# Autodesk Inventor assembly: Chassis assembly
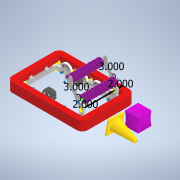
[picture p0: Inventor's stored thumbnail of the model, 180x180]
Saved by Autodesk Inventor 2022 (Build 260153000, 153)
## iProperties
Created: 2022-11-14
Part Number: Chassis assembly
Document SubType Name: Assembly
Designer: s135320
Author: s135320
## Documents named in this file (35)
- D:\Chassis assembly.iam
- D:\Chassis\Chassis side 1.ipt
- D:\Chassis\Chassis side 2.ipt
- D:\STEP Files\Hardware\Gussets\TTB T Gusset\TTB-00012_T-Gusset.ipt
- D:\STEP Files\Bearings\1-2inch Hex Bering\217-3875-STEP-20140818.ipt
- D:\STEP Files\Gearboxes\WCP SS Flipped Gearbox\WCP-0235.iam
- D:\bumper simple.ipt
- D:\bumper bracket.ipt
- D:\1872A111_Slide-Snap Draw Latch.ipt
- D:\bumper bracket - Copy.ipt
- D:\drive hex shaft.ipt
- D:\bumper piece 1.ipt
- D:\Drive spacer.ipt
- D:\WCP-0087.ipt
- D:\STEP Files\Hardware\Shaft Collars\TTB Balanced Hex Collar\TTB-0013_Balanced Half Inch Hex Shaft Collar.ipt
- D:\bumper beam.ipt
- D:\STEP Files\Hardware\teleiscope arm\WCP - Greyt Telescope (Stages 1-4).iam
- D:\Imported Components\am-0940b 6 in HiGrip Wheel\am-0940b 6 in HiGrip Wheel.iam
- D:\Imported Components\am-2568 500EX Hex Hub\am-2568 500EX Hex Hub.ipt
- D:\Robot bottom.ipt
- D:\STEP Files\Electrical\Breaker\am-0282 120a Circuit Breaker.ipt
- D:\STEP Files\Electrical\Power Distribution Hub\REV-11-1850.ipt
- D:\STEP Files\Electrical\Pneumatic Hub\REV-11-1852.ipt
- D:\STEP Files\Electrical\Roborio V2\am-3000a National Instruments roboRIO 2.ipt
- D:\STEP Files\Pnumatics\Compressor\am-3227 Pneumatic Compressor 1.1_Pump REV2.ipt
- D:\STEP Files\Electrical\Battery\ELEC_Battery_NP18-12B.iam
- D:\Intake hex.ipt
- D:\intake-1.ipt
- D:\TTB-0058 5M 15t HTD ALUMINUM PULLEY.ipt
- D:\am-3480 4IN 500Hex Bore Compliant Wheel REV2.ipt
- D:\am-4541 Sushi Roller 500 Hex Bore.ipt
- D:\Intake mount.ipt
- D:\Intake base hex.ipt
- D:\Imported Components\am-4700_bpc Cube\am-4700_bpc Cube.ipt
- D:\Imported Components\am-4700_syc Cone\am-4700_syc Cone.ipt
## Components (171 placed, 34 different names)
1. WCP - Greyt Telescope (Stages 1-4):1 [sub-assembly]
2. bumper simple:1 — Mate:69, Mate:70, Flush:10, Mate:83, Mate:86, Mate:98, Mate:104, Mate:303, Mate:354, Mate:355, Mate:356, Mate:357, Mate:358, Mate:412
3. Intake base hex:1 — Mate:532, Mate:533, Mate:534, Mate:535, Mate:536
4. 217-3875-STEP-20140818:30 — Mate:528, Mate:529, Mate:534
5. 217-3875-STEP-20140818:31 — Mate:530, Mate:531, Mate:532, Mate:533
6. am-4700_bpc Cube:1
7. am-4700_syc Cone:1
8. 217-3875-STEP-20140818:29 — Mate:525, Mate:526
9. 217-3875-STEP-20140818:28 — Mate:524, Mate:527, Mate:535, Mate:536
10. 217-3875-STEP-20140818:27 — Mate:521, Mate:522
11. 217-3875-STEP-20140818:26 — Mate:520, Mate:523
12. Intake mount:2 — Mate:517, Mate:518, Mate:519, Mate:524, Mate:525, Mate:526, Mate:527
13. Intake mount:1 — Mate:514, Mate:515, Mate:516, Mate:520, Mate:521, Mate:522, Mate:523, Mate:537
14. Chassis side 1:1 — Mate:8, Mate:9, Flush:3, Mate:10, Mate:11, Flush:4, Mate:22, Mate:29, Mate:30, Mate:31, Mate:32, Mate:37, Mate:38, Mate:39, Mate:40, Mate:41, Mate:42, Mate:45, Mate:55, Mate:61, Mate:64, Mate:65, Mate:68, Mate:126, Mate:200, Mate:287, Mate:288, Mate:331, Mate:332, Mate:333, Mate:348, Mate:349, Mate:350, Mate:351, Mate:352, Mate:353
15. Chassis side 1:2 — Mate:1, Mate:2, Mate:3, Mate:14, Mate:15, Flush:6, Mate:20, Mate:25, Mate:26, Mate:27, Mate:28, Mate:33, Mate:34, Mate:35, Mate:36, Mate:43, Mate:44, Mate:46, Mate:56, Mate:62, Mate:63, Mate:279, Mate:280, Mate:292, Mate:293, Mate:294, Mate:295, Mate:325, Mate:326, Mate:327, Mate:328, Mate:329, Mate:330, Mate:410, Mate:411
16. Chassis side 2:1 — Mate:12, Mate:13, Flush:5, Mate:21, Flush:9, Mate:23, Mate:24, Mate:57, Mate:58, Mate:59, Mate:60, Mate:69, Mate:70, Mate:87, Mate:88, Mate:99, Mate:100, Mate:291
17. Chassis side 2:2 — Mate:4, Mate:5, Flush:1, Mate:6, Mate:7, Flush:2, Mate:18, Mate:19, Flush:8, Flush:10, Mate:84, Mate:85, Mate:105, Mate:106, Mate:290, Mate:407, Mate:408, Mate:409
18. TTB-00012_T-Gusset:1 — Mate:14, Mate:15, Flush:6, Mate:57
19. TTB-00012_T-Gusset:2 — Mate:1, Mate:2, Mate:3, Mate:4, Mate:5, Flush:1, Mate:56, Mate:407, Mate:517, Mate:518, Mate:519
20. TTB-00012_T-Gusset:3 — Mate:22, Mate:23, Mate:24, Mate:60, Mate:61
21. TTB-00012_T-Gusset:5 — Mate:20, Mate:21, Flush:9, Mate:58, Mate:59
22. TTB-00012_T-Gusset:6 — Mate:6, Mate:7, Flush:2, Mate:8, Mate:9, Flush:3, Mate:55, Mate:290, Mate:514, Mate:515, Mate:516
23. TTB-00012_T-Gusset:7 — Mate:10, Mate:11, Flush:4, Mate:12, Mate:13, Flush:5, Mate:291
24. TTB-00012_T-Gusset:8 — Mate:18, Mate:19, Flush:8
25. 217-3875-STEP-20140818:3 — Mate:37, Mate:38, Mate:197, Mate:198, Mate:406
26. 217-3875-STEP-20140818:4 — Mate:29, Mate:30, Mate:200, Mate:201
27. 217-3875-STEP-20140818:5 — Mate:39, Mate:40, Mate:203, Mate:204, Mate:388
28. 217-3875-STEP-20140818:6 — Mate:35, Mate:36, Mate:208
29. 217-3875-STEP-20140818:8 — Mate:33, Mate:34, Mate:252, Mate:253, Mate:254
30. 217-3875-STEP-20140818:9 — Mate:31, Mate:32, Mate:202
31. 217-3875-STEP-20140818:11 — Mate:27, Mate:28, Mate:385
32. 217-3875-STEP-20140818:12 — Mate:25, Mate:26, Mate:206, Mate:207, Mate:379
33. WCP-0235:1 [sub-assembly] — Mate:43, Mate:44, Mate:46, Mate:362, Mate:364
34. WCP-0235:2 [sub-assembly] — Mate:41, Mate:42, Mate:45, Mate:401, Mate:402
35. 217-3875-STEP-20140818:13 — Mate:62, Mate:63, Mate:382
36. 217-3875-STEP-20140818:14 — Mate:64, Mate:65, Mate:107, Mate:108, Mate:111
37. 217-3875-STEP-20140818:16 — Mate:68, Mate:126, Mate:400
38. bumper bracket:6 — Mate:86, Mate:87
39. 1872A111_Slide-Snap Draw Latch:6 — Mate:88
40. bumper bracket:7 — Mate:83, Mate:85
41. 1872A111_Slide-Snap Draw Latch:7 — Mate:84
42. 1872A111_Slide-Snap Draw Latch:8 — Mate:99
43. bumper bracket - Copy:3 — Mate:98, Mate:100
44. 1872A111_Slide-Snap Draw Latch:9 — Mate:105, Mate:465
45. bumper bracket - Copy:4 — Mate:104, Mate:106, Mate:465
46. drive hex shaft:1 — Mate:107, Mate:108, Mate:109, Mate:110, Mate:112, Mate:113, Mate:115, Mate:116, Flush:11, Mate:398, Mate:399
47. bumper piece 1:1 — Mate:292, Mate:293, Mate:294, Mate:295, Mate:296, Mate:297
48. Drive spacer:1 — Mate:109, Mate:110, Mate:111, Mate:114
49. WCP-0087:1 — Mate:112, Mate:113, Mate:114, Mate:139
50. TTB-0013_Balanced Half Inch Hex Shaft Collar:1 — Mate:115, Mate:116, Flush:11, Mate:139
51. drive hex shaft:2 — Mate:197, Mate:198, Mate:404, Mate:405
52. Drive spacer:3 — Mate:201
53. WCP-0087:2
54. TTB-0013_Balanced Half Inch Hex Shaft Collar:3
55. drive hex shaft:3 — Mate:203, Mate:204, Mate:386, Mate:387
56. Drive spacer:5 — Mate:202
57. WCP-0087:3
58. TTB-0013_Balanced Half Inch Hex Shaft Collar:5
59. drive hex shaft:4 — Mate:206, Mate:207, Mate:377, Mate:378, Flush:19
60. Drive spacer:7 — Mate:208
61. WCP-0087:4
62. TTB-0013_Balanced Half Inch Hex Shaft Collar:7 — Flush:19
63. drive hex shaft:5 — Mate:380, Mate:381, Flush:18
64. Drive spacer:9
65. WCP-0087:5
66. TTB-0013_Balanced Half Inch Hex Shaft Collar:9 — Flush:18
67. drive hex shaft:6 — Mate:252, Mate:253, Mate:383, Mate:384, Flush:17
68. Drive spacer:11 — Mate:254
69. WCP-0087:6
70. TTB-0013_Balanced Half Inch Hex Shaft Collar:11 — Flush:17
71. 217-3875-STEP-20140818:17 — Mate:279, Mate:280, Mate:363
72. 217-3875-STEP-20140818:18 — Mate:287, Mate:288, Mate:403
73. bumper beam:1 — Mate:296, Mate:297, Mate:301, Mate:302
74. 1872A111_Slide-Snap Draw Latch:10 — Mate:301
75. bumper bracket - Copy:5 — Mate:302, Mate:303
76. bumper piece 1:2 — Mate:325, Mate:326
77. bumper beam:2 — Mate:327
78. 1872A111_Slide-Snap Draw Latch:11
79. bumper bracket - Copy:6 — Mate:357
80. bumper piece 1:3 — Mate:328, Mate:329
81. bumper beam:3 — Mate:330
82. 1872A111_Slide-Snap Draw Latch:12
83. bumper bracket - Copy:7 — Mate:358
84. bumper piece 1:4 — Mate:331, Mate:332
85. bumper beam:4 — Mate:333
86. 1872A111_Slide-Snap Draw Latch:13
87. bumper bracket - Copy:8 — Mate:354
88. bumper piece 1:5 — Mate:348, Mate:349
89. bumper beam:5 — Mate:350
90. 1872A111_Slide-Snap Draw Latch:14
91. bumper bracket - Copy:9 — Mate:355
92. bumper piece 1:6 — Mate:351, Mate:352
93. bumper beam:6 — Mate:353
94. 1872A111_Slide-Snap Draw Latch:15
95. bumper bracket - Copy:10 — Mate:356
96. am-0940b 6 in HiGrip Wheel:10 [sub-assembly] — Mate:359, Mate:360, Mate:361
97. am-2568 500EX Hex Hub:9 — Mate:359, Mate:360, Mate:361, Mate:362, Mate:363, Mate:364
98. am-0940b 6 in HiGrip Wheel:11 [sub-assembly]
99. am-2568 500EX Hex Hub:10 — Mate:380, Mate:381, Mate:382
100. am-0940b 6 in HiGrip Wheel:12 [sub-assembly]
101. am-2568 500EX Hex Hub:11 — Mate:377, Mate:378, Mate:379
102. am-0940b 6 in HiGrip Wheel:13 [sub-assembly]
103. am-2568 500EX Hex Hub:12 — Mate:383, Mate:384, Mate:385
104. am-0940b 6 in HiGrip Wheel:14 [sub-assembly]
105. am-2568 500EX Hex Hub:13 — Mate:386, Mate:387, Mate:388
106. am-0940b 6 in HiGrip Wheel:15 [sub-assembly]
107. am-2568 500EX Hex Hub:14 — Mate:401, Mate:402, Mate:403
108. am-0940b 6 in HiGrip Wheel:16 [sub-assembly]
109. am-2568 500EX Hex Hub:15 — Mate:398, Mate:399, Mate:400
110. am-0940b 6 in HiGrip Wheel:17 [sub-assembly]
111. am-2568 500EX Hex Hub:16 — Mate:404, Mate:405, Mate:406
112. TTB-00012_T-Gusset:9 — Mate:408, Mate:409, Mate:410
113. ELEC_Battery_NP18-12B:1 [sub-assembly]
114. am-3227 Pneumatic Compressor 1.1_Pump REV2:1 — Mate:418
115. am-3000a National Instruments roboRIO 2:1 — Mate:413
116. Robot bottom:1 — Mate:411, Mate:412, Mate:413, Mate:415, Mate:416, Mate:417, Mate:418
117. am-0282 120a Circuit Breaker:1 — Mate:417
118. REV-11-1852:1 — Mate:416
119. REV-11-1850:1 — Mate:415
120. TTB-0013_Balanced Half Inch Hex Shaft Collar:15 — Mate:490, Mate:491, Mate:500
121. am-4541 Sushi Roller 500 Hex Bore:32 — Mate:492, Mate:493, Mate:494, Mate:495, Mate:501
122. TTB-0013_Balanced Half Inch Hex Shaft Collar:16 — Mate:497, Mate:498, Mate:499, Flush:22
123. 217-3875-STEP-20140818:25 — Mate:480, Mate:481, Mate:484, Mate:485, Mate:486, Mate:487, Mate:496, Mate:500
124. 217-3875-STEP-20140818:24 — Mate:479, Mate:482, Mate:483, Mate:495, Mate:499, Mate:511, Mate:512
125. am-4541 Sushi Roller 500 Hex Bore:2 — Mate:508, Mate:509, Mate:510
126. intake-1:3 — Mate:479, Mate:480, Mate:481, Mate:482, Mate:486, Mate:487, Mate:501, Mate:510, Mate:512, Mate:530, Mate:531, Mate:537
127. TTB-0013_Balanced Half Inch Hex Shaft Collar:13 — Mate:442, Mate:443, Flush:21, Mate:444
128. TTB-0013_Balanced Half Inch Hex Shaft Collar:12 — Mate:440, Mate:441, Flush:20, Mate:445, Mate:472
129. TTB-0058 5M 15t HTD ALUMINUM PULLEY:2 — Mate:436, Mate:437, Mate:438, Mate:444
130. TTB-0058 5M 15t HTD ALUMINUM PULLEY:1 — Mate:434, Mate:435, Mate:439, Mate:445
131. 217-3875-STEP-20140818:23 — Mate:433, Mate:439, Mate:469, Mate:472, Mate:513
132. 217-3875-STEP-20140818:22 — Mate:431, Mate:432, Mate:438, Mate:475
133. intake-1:2 — Mate:507, Mate:528, Mate:529
134. Intake hex:2 — Mate:433, Mate:434, Mate:435, Mate:440, Mate:441, Flush:20, Mate:469, Mate:484, Mate:485, Mate:490, Mate:491, Mate:496, Mate:502, Mate:503, Mate:504, Mate:505, Mate:508, Mate:509, Mate:513
135. Intake hex:1 — Mate:431, Mate:432, Mate:436, Mate:437, Mate:442, Mate:443, Flush:21, Mate:473, Mate:474, Mate:476, Mate:477, Mate:483, Mate:492, Mate:493, Mate:497, Mate:498, Mate:511, Flush:22
136. am-4541 Sushi Roller 500 Hex Bore:33 — Mate:502, Mate:503, Mate:506, Mate:507
137. am-3480 4IN 500Hex Bore Compliant Wheel REV2:33 — Mate:504, Mate:505, Mate:506
138. am-4541 Sushi Roller 500 Hex Bore:34
139. am-3480 4IN 500Hex Bore Compliant Wheel REV2:34
140. am-4541 Sushi Roller 500 Hex Bore:35
141. am-3480 4IN 500Hex Bore Compliant Wheel REV2:35
142. am-4541 Sushi Roller 500 Hex Bore:36
143. am-3480 4IN 500Hex Bore Compliant Wheel REV2:36
144. am-4541 Sushi Roller 500 Hex Bore:37
145. am-3480 4IN 500Hex Bore Compliant Wheel REV2:37
146. am-4541 Sushi Roller 500 Hex Bore:38
147. am-3480 4IN 500Hex Bore Compliant Wheel REV2:38
148. am-4541 Sushi Roller 500 Hex Bore:39
149. am-3480 4IN 500Hex Bore Compliant Wheel REV2:39
150. am-4541 Sushi Roller 500 Hex Bore:40
151. am-3480 4IN 500Hex Bore Compliant Wheel REV2:40
152. am-4541 Sushi Roller 500 Hex Bore:41
153. am-3480 4IN 500Hex Bore Compliant Wheel REV2:41
154. am-3480 4IN 500Hex Bore Compliant Wheel REV2:8 — Mate:476, Mate:477, Mate:478
155. am-4541 Sushi Roller 500 Hex Bore:23 — Mate:473, Mate:474, Mate:475, Mate:478
156. am-3480 4IN 500Hex Bore Compliant Wheel REV2:25
157. am-4541 Sushi Roller 500 Hex Bore:24
158. am-3480 4IN 500Hex Bore Compliant Wheel REV2:26
159. am-4541 Sushi Roller 500 Hex Bore:25
160. am-3480 4IN 500Hex Bore Compliant Wheel REV2:27
161. am-4541 Sushi Roller 500 Hex Bore:26
162. am-3480 4IN 500Hex Bore Compliant Wheel REV2:28
163. am-4541 Sushi Roller 500 Hex Bore:27
164. am-3480 4IN 500Hex Bore Compliant Wheel REV2:29
165. am-4541 Sushi Roller 500 Hex Bore:28
166. am-3480 4IN 500Hex Bore Compliant Wheel REV2:30
167. am-4541 Sushi Roller 500 Hex Bore:29
168. am-3480 4IN 500Hex Bore Compliant Wheel REV2:31
169. am-4541 Sushi Roller 500 Hex Bore:30
170. am-3480 4IN 500Hex Bore Compliant Wheel REV2:32 — Mate:494
171. am-4541 Sushi Roller 500 Hex Bore:31
## Component patterns: (9 elements, first: am-4541 Sushi Roller 500 Hex Bore:33 + am-3480 4IN 500Hex Bore Compliant Wheel REV2:33), (9 elements, first: am-3480 4IN 500Hex Bore Compliant Wheel REV2:8 + am-4541 Sushi Roller 500 Hex Bore:23)
## Relationships (385: Mate 364, Flush 21)
- Mate:1: Chassis side 1:2 ↔ TTB-00012_T-Gusset:2
- Mate:2: Chassis side 1:2 ↔ TTB-00012_T-Gusset:2
- Mate:3: Chassis side 1:2 ↔ TTB-00012_T-Gusset:2
- Mate:4: Chassis side 2:2 ↔ TTB-00012_T-Gusset:2
- Mate:5: Chassis side 2:2 ↔ TTB-00012_T-Gusset:2
- Flush:1: Chassis side 2:2 ↔ TTB-00012_T-Gusset:2
- Mate:6: Chassis side 2:2 ↔ TTB-00012_T-Gusset:6
- Mate:7: Chassis side 2:2 ↔ TTB-00012_T-Gusset:6
- Flush:2: Chassis side 2:2 ↔ TTB-00012_T-Gusset:6
- Mate:8: Chassis side 1:1 ↔ TTB-00012_T-Gusset:6
- Mate:9: Chassis side 1:1 ↔ TTB-00012_T-Gusset:6
- Flush:3: Chassis side 1:1 ↔ TTB-00012_T-Gusset:6
- Mate:10: Chassis side 1:1 ↔ TTB-00012_T-Gusset:7
- Mate:11: Chassis side 1:1 ↔ TTB-00012_T-Gusset:7
- Flush:4: Chassis side 1:1 ↔ TTB-00012_T-Gusset:7
- Mate:12: Chassis side 2:1 ↔ TTB-00012_T-Gusset:7
- Mate:13: Chassis side 2:1 ↔ TTB-00012_T-Gusset:7
- Flush:5: Chassis side 2:1 ↔ TTB-00012_T-Gusset:7
- Mate:14: Chassis side 1:2 ↔ TTB-00012_T-Gusset:1
- Mate:15: Chassis side 1:2 ↔ TTB-00012_T-Gusset:1
- Flush:6: Chassis side 1:2 ↔ TTB-00012_T-Gusset:1
- Mate:18: Chassis side 2:2 ↔ TTB-00012_T-Gusset:8
- Mate:19: Chassis side 2:2 ↔ TTB-00012_T-Gusset:8
- Flush:8: Chassis side 2:2 ↔ TTB-00012_T-Gusset:8
- Mate:20: Chassis side 1:2 ↔ TTB-00012_T-Gusset:5
- Mate:21: Chassis side 2:1 ↔ TTB-00012_T-Gusset:5
- Flush:9: Chassis side 2:1 ↔ TTB-00012_T-Gusset:5
- Mate:22: Chassis side 1:1 ↔ TTB-00012_T-Gusset:3
- Mate:23: Chassis side 2:1 ↔ TTB-00012_T-Gusset:3
- Mate:24: Chassis side 2:1 ↔ TTB-00012_T-Gusset:3
- Mate:25: Chassis side 1:2 ↔ 217-3875-STEP-20140818:12
- Mate:26: Chassis side 1:2 ↔ 217-3875-STEP-20140818:12
- Mate:27: Chassis side 1:2 ↔ 217-3875-STEP-20140818:11
- Mate:28: Chassis side 1:2 ↔ 217-3875-STEP-20140818:11
- Mate:29: Chassis side 1:1 ↔ 217-3875-STEP-20140818:4
- Mate:30: Chassis side 1:1 ↔ 217-3875-STEP-20140818:4
- Mate:31: Chassis side 1:1 ↔ 217-3875-STEP-20140818:9
- Mate:32: Chassis side 1:1 ↔ 217-3875-STEP-20140818:9
- Mate:33: Chassis side 1:2 ↔ 217-3875-STEP-20140818:8
- Mate:34: Chassis side 1:2 ↔ 217-3875-STEP-20140818:8
- Mate:35: Chassis side 1:2 ↔ 217-3875-STEP-20140818:6
- Mate:36: Chassis side 1:2 ↔ 217-3875-STEP-20140818:6
- Mate:37: Chassis side 1:1 ↔ 217-3875-STEP-20140818:3
- Mate:38: Chassis side 1:1 ↔ 217-3875-STEP-20140818:3
- Mate:39: Chassis side 1:1 ↔ 217-3875-STEP-20140818:5
- Mate:40: Chassis side 1:1 ↔ 217-3875-STEP-20140818:5
- Mate:41: Chassis side 1:1 ↔ WCP-0235:2
- Mate:42: Chassis side 1:1 ↔ WCP-0235:2
- Mate:43: Chassis side 1:2 ↔ WCP-0235:1
- Mate:44: Chassis side 1:2 ↔ WCP-0235:1
- Mate:45: Chassis side 1:1 ↔ WCP-0235:2
- Mate:46: Chassis side 1:2 ↔ WCP-0235:1
- Mate:55: Chassis side 1:1 ↔ TTB-00012_T-Gusset:6
- Mate:56: Chassis side 1:2 ↔ TTB-00012_T-Gusset:2
- Mate:57: Chassis side 2:1 ↔ TTB-00012_T-Gusset:1
- Mate:58: Chassis side 2:1 ↔ TTB-00012_T-Gusset:5
- Mate:59: Chassis side 2:1 ↔ TTB-00012_T-Gusset:5
- Mate:60: Chassis side 2:1 ↔ TTB-00012_T-Gusset:3
- Mate:61: Chassis side 1:1 ↔ TTB-00012_T-Gusset:3
- Mate:62: Chassis side 1:2 ↔ 217-3875-STEP-20140818:13
- Mate:63: Chassis side 1:2 ↔ 217-3875-STEP-20140818:13
- Mate:64: Chassis side 1:1 ↔ 217-3875-STEP-20140818:14
- Mate:65: Chassis side 1:1 ↔ 217-3875-STEP-20140818:14
- Mate:68: Chassis side 1:1 ↔ 217-3875-STEP-20140818:16
- Mate:69: bumper simple:1 ↔ Chassis side 2:1
- Mate:70: bumper simple:1 ↔ Chassis side 2:1
- Flush:10: bumper simple:1 ↔ Chassis side 2:2
- [Mate]: bumper bracket:6 ↔ 1872A111_Slide-Snap Draw Latch:6
- [Mate]: bumper bracket:6 ↔ 1872A111_Slide-Snap Draw Latch:6
- [Mate]: bumper bracket:6 ↔ 1872A111_Slide-Snap Draw Latch:6
- [Mate]: bumper bracket:7 ↔ 1872A111_Slide-Snap Draw Latch:7
- [Mate]: bumper bracket:7 ↔ 1872A111_Slide-Snap Draw Latch:7
- [Mate]: bumper bracket:7 ↔ 1872A111_Slide-Snap Draw Latch:7
- Mate:83: bumper simple:1 ↔ bumper bracket:7
- Mate:84: Chassis side 2:2 ↔ 1872A111_Slide-Snap Draw Latch:7
- Mate:85: Chassis side 2:2 ↔ bumper bracket:7
- Mate:86: bumper simple:1 ↔ bumper bracket:6
- Mate:87: Chassis side 2:1 ↔ bumper bracket:6
- Mate:88: Chassis side 2:1 ↔ 1872A111_Slide-Snap Draw Latch:6
- [Mate]: 1872A111_Slide-Snap Draw Latch:8 ↔ bumper bracket - Copy:3
- [Mate]: 1872A111_Slide-Snap Draw Latch:8 ↔ bumper bracket - Copy:3
- [Mate]: 1872A111_Slide-Snap Draw Latch:8 ↔ bumper bracket - Copy:3
- Mate:98: bumper simple:1 ↔ bumper bracket - Copy:3
- Mate:99: Chassis side 2:1 ↔ 1872A111_Slide-Snap Draw Latch:8
- Mate:100: Chassis side 2:1 ↔ bumper bracket - Copy:3
- [Mate]: 1872A111_Slide-Snap Draw Latch:9 ↔ bumper bracket - Copy:4
- [Mate]: 1872A111_Slide-Snap Draw Latch:9 ↔ bumper bracket - Copy:4
- [Mate]: 1872A111_Slide-Snap Draw Latch:9 ↔ bumper bracket - Copy:4
- Mate:104: bumper simple:1 ↔ bumper bracket - Copy:4
- Mate:105: Chassis side 2:2 ↔ 1872A111_Slide-Snap Draw Latch:9
- Mate:106: Chassis side 2:2 ↔ bumper bracket - Copy:4
- Mate:107: 217-3875-STEP-20140818:14 ↔ drive hex shaft:1
- Mate:108: 217-3875-STEP-20140818:14 ↔ drive hex shaft:1
- Mate:109: drive hex shaft:1 ↔ Drive spacer:1
- Mate:110: drive hex shaft:1 ↔ Drive spacer:1
- Mate:111: 217-3875-STEP-20140818:14 ↔ Drive spacer:1
- Mate:112: drive hex shaft:1 ↔ WCP-0087:1
- Mate:113: drive hex shaft:1 ↔ WCP-0087:1
- Mate:114: Drive spacer:1 ↔ WCP-0087:1
- Mate:115: drive hex shaft:1 ↔ TTB-0013_Balanced Half Inch Hex Shaft Collar:1
- Mate:116: drive hex shaft:1 ↔ TTB-0013_Balanced Half Inch Hex Shaft Collar:1
- Flush:11: drive hex shaft:1 ↔ TTB-0013_Balanced Half Inch Hex Shaft Collar:1
- Mate:126: Chassis side 1:1 ↔ 217-3875-STEP-20140818:16
- Mate:139: WCP-0087:1 ↔ TTB-0013_Balanced Half Inch Hex Shaft Collar:1
- [Mate]: drive hex shaft:2 ↔ Drive spacer:3
- [Mate]: drive hex shaft:2 ↔ Drive spacer:3
- [Mate]: drive hex shaft:2 ↔ WCP-0087:2
- [Mate]: drive hex shaft:2 ↔ WCP-0087:2
- [Mate]: Drive spacer:3 ↔ WCP-0087:2
- [Mate]: drive hex shaft:2 ↔ TTB-0013_Balanced Half Inch Hex Shaft Collar:3
- [Mate]: drive hex shaft:2 ↔ TTB-0013_Balanced Half Inch Hex Shaft Collar:3
- [Flush]: drive hex shaft:2 ↔ TTB-0013_Balanced Half Inch Hex Shaft Collar:3
- [Mate]: WCP-0087:2 ↔ TTB-0013_Balanced Half Inch Hex Shaft Collar:3
- [Mate]: drive hex shaft:3 ↔ Drive spacer:5
- [Mate]: drive hex shaft:3 ↔ Drive spacer:5
- [Mate]: drive hex shaft:3 ↔ WCP-0087:3
- [Mate]: drive hex shaft:3 ↔ WCP-0087:3
- [Mate]: Drive spacer:5 ↔ WCP-0087:3
- [Mate]: drive hex shaft:3 ↔ TTB-0013_Balanced Half Inch Hex Shaft Collar:5
- [Mate]: drive hex shaft:3 ↔ TTB-0013_Balanced Half Inch Hex Shaft Collar:5
- [Flush]: drive hex shaft:3 ↔ TTB-0013_Balanced Half Inch Hex Shaft Collar:5
- [Mate]: WCP-0087:3 ↔ TTB-0013_Balanced Half Inch Hex Shaft Collar:5
- [Mate]: drive hex shaft:4 ↔ Drive spacer:7
- [Mate]: drive hex shaft:4 ↔ Drive spacer:7
- [Mate]: drive hex shaft:4 ↔ WCP-0087:4
- [Mate]: drive hex shaft:4 ↔ WCP-0087:4
- [Mate]: Drive spacer:7 ↔ WCP-0087:4
- [Mate]: drive hex shaft:4 ↔ TTB-0013_Balanced Half Inch Hex Shaft Collar:7
- [Mate]: drive hex shaft:4 ↔ TTB-0013_Balanced Half Inch Hex Shaft Collar:7
- [Flush]: drive hex shaft:4 ↔ TTB-0013_Balanced Half Inch Hex Shaft Collar:7
- [Mate]: WCP-0087:4 ↔ TTB-0013_Balanced Half Inch Hex Shaft Collar:7
- Mate:197: 217-3875-STEP-20140818:3 ↔ drive hex shaft:2
- Mate:198: 217-3875-STEP-20140818:3 ↔ drive hex shaft:2
- Mate:200: Chassis side 1:1 ↔ 217-3875-STEP-20140818:4
- Mate:201: 217-3875-STEP-20140818:4 ↔ Drive spacer:3
- Mate:202: 217-3875-STEP-20140818:9 ↔ Drive spacer:5
- Mate:203: 217-3875-STEP-20140818:5 ↔ drive hex shaft:3
- Mate:204: 217-3875-STEP-20140818:5 ↔ drive hex shaft:3
- Mate:206: 217-3875-STEP-20140818:12 ↔ drive hex shaft:4
- Mate:207: 217-3875-STEP-20140818:12 ↔ drive hex shaft:4
- Mate:208: 217-3875-STEP-20140818:6 ↔ Drive spacer:7
- [Mate]: drive hex shaft:5 ↔ Drive spacer:9
- [Mate]: drive hex shaft:5 ↔ Drive spacer:9
- [Mate]: drive hex shaft:5 ↔ WCP-0087:5
- [Mate]: drive hex shaft:5 ↔ WCP-0087:5
- [Mate]: Drive spacer:9 ↔ WCP-0087:5
- [Mate]: drive hex shaft:5 ↔ TTB-0013_Balanced Half Inch Hex Shaft Collar:9
- [Mate]: drive hex shaft:5 ↔ TTB-0013_Balanced Half Inch Hex Shaft Collar:9
- [Flush]: drive hex shaft:5 ↔ TTB-0013_Balanced Half Inch Hex Shaft Collar:9
- [Mate]: WCP-0087:5 ↔ TTB-0013_Balanced Half Inch Hex Shaft Collar:9
- [Mate]: drive hex shaft:6 ↔ Drive spacer:11
- [Mate]: drive hex shaft:6 ↔ Drive spacer:11
- [Mate]: drive hex shaft:6 ↔ WCP-0087:6
- [Mate]: drive hex shaft:6 ↔ WCP-0087:6
- [Mate]: Drive spacer:11 ↔ WCP-0087:6
- [Mate]: drive hex shaft:6 ↔ TTB-0013_Balanced Half Inch Hex Shaft Collar:11
- [Mate]: drive hex shaft:6 ↔ TTB-0013_Balanced Half Inch Hex Shaft Collar:11
- [Flush]: drive hex shaft:6 ↔ TTB-0013_Balanced Half Inch Hex Shaft Collar:11
- [Mate]: WCP-0087:6 ↔ TTB-0013_Balanced Half Inch Hex Shaft Collar:11
- Mate:252: 217-3875-STEP-20140818:8 ↔ drive hex shaft:6
- Mate:253: 217-3875-STEP-20140818:8 ↔ drive hex shaft:6
- Mate:254: 217-3875-STEP-20140818:8 ↔ Drive spacer:11
- Mate:279: Chassis side 1:2 ↔ 217-3875-STEP-20140818:17
- Mate:280: Chassis side 1:2 ↔ 217-3875-STEP-20140818:17
- Mate:287: Chassis side 1:1 ↔ 217-3875-STEP-20140818:18
- Mate:288: Chassis side 1:1 ↔ 217-3875-STEP-20140818:18
- Mate:290: Chassis side 2:2 ↔ TTB-00012_T-Gusset:6
- Mate:291: Chassis side 2:1 ↔ TTB-00012_T-Gusset:7
- Mate:292: Chassis side 1:2 ↔ bumper piece 1:1
- Mate:293: Chassis side 1:2 ↔ bumper piece 1:1
- Mate:294: Chassis side 1:2 ↔ bumper piece 1:1
- Mate:295: Chassis side 1:2 ↔ bumper piece 1:1
- Mate:296: bumper piece 1:1 ↔ bumper beam:1
- Mate:297: bumper piece 1:1 ↔ bumper beam:1
- [Mate]: 1872A111_Slide-Snap Draw Latch:10 ↔ bumper bracket - Copy:5
- [Mate]: 1872A111_Slide-Snap Draw Latch:10 ↔ bumper bracket - Copy:5
- [Mate]: 1872A111_Slide-Snap Draw Latch:10 ↔ bumper bracket - Copy:5
- Mate:301: bumper beam:1 ↔ 1872A111_Slide-Snap Draw Latch:10
- Mate:302: bumper beam:1 ↔ bumper bracket - Copy:5
- Mate:303: bumper simple:1 ↔ bumper bracket - Copy:5
- [Mate]: bumper piece 1:2 ↔ bumper beam:2
- [Mate]: bumper piece 1:2 ↔ bumper beam:2
- [Mate]: 1872A111_Slide-Snap Draw Latch:11 ↔ bumper bracket - Copy:6
- [Mate]: 1872A111_Slide-Snap Draw Latch:11 ↔ bumper bracket - Copy:6
- [Mate]: 1872A111_Slide-Snap Draw Latch:11 ↔ bumper bracket - Copy:6
- [Mate]: bumper beam:2 ↔ 1872A111_Slide-Snap Draw Latch:11
- [Mate]: bumper beam:2 ↔ bumper bracket - Copy:6
- [Mate]: bumper piece 1:3 ↔ bumper beam:3
- [Mate]: bumper piece 1:3 ↔ bumper beam:3
- [Mate]: 1872A111_Slide-Snap Draw Latch:12 ↔ bumper bracket - Copy:7
- [Mate]: 1872A111_Slide-Snap Draw Latch:12 ↔ bumper bracket - Copy:7
- [Mate]: 1872A111_Slide-Snap Draw Latch:12 ↔ bumper bracket - Copy:7
- [Mate]: bumper beam:3 ↔ 1872A111_Slide-Snap Draw Latch:12
- [Mate]: bumper beam:3 ↔ bumper bracket - Copy:7
- [Mate]: bumper piece 1:4 ↔ bumper beam:4
- [Mate]: bumper piece 1:4 ↔ bumper beam:4
- [Mate]: 1872A111_Slide-Snap Draw Latch:13 ↔ bumper bracket - Copy:8
- [Mate]: 1872A111_Slide-Snap Draw Latch:13 ↔ bumper bracket - Copy:8
- [Mate]: 1872A111_Slide-Snap Draw Latch:13 ↔ bumper bracket - Copy:8
- [Mate]: bumper beam:4 ↔ 1872A111_Slide-Snap Draw Latch:13
- [Mate]: bumper beam:4 ↔ bumper bracket - Copy:8
- Mate:325: Chassis side 1:2 ↔ bumper piece 1:2
- Mate:326: Chassis side 1:2 ↔ bumper piece 1:2
- Mate:327: Chassis side 1:2 ↔ bumper beam:2
- Mate:328: Chassis side 1:2 ↔ bumper piece 1:3
- Mate:329: Chassis side 1:2 ↔ bumper piece 1:3
- Mate:330: Chassis side 1:2 ↔ bumper beam:3
- Mate:331: Chassis side 1:1 ↔ bumper piece 1:4
- Mate:332: Chassis side 1:1 ↔ bumper piece 1:4
- Mate:333: Chassis side 1:1 ↔ bumper beam:4
- [Mate]: bumper piece 1:5 ↔ bumper beam:5
- [Mate]: bumper piece 1:5 ↔ bumper beam:5
- [Mate]: 1872A111_Slide-Snap Draw Latch:14 ↔ bumper bracket - Copy:9
- [Mate]: 1872A111_Slide-Snap Draw Latch:14 ↔ bumper bracket - Copy:9
- [Mate]: 1872A111_Slide-Snap Draw Latch:14 ↔ bumper bracket - Copy:9
- [Mate]: bumper beam:5 ↔ 1872A111_Slide-Snap Draw Latch:14
- [Mate]: bumper beam:5 ↔ bumper bracket - Copy:9
- [Mate]: bumper piece 1:6 ↔ bumper beam:6
- [Mate]: bumper piece 1:6 ↔ bumper beam:6
- [Mate]: 1872A111_Slide-Snap Draw Latch:15 ↔ bumper bracket - Copy:10
- [Mate]: 1872A111_Slide-Snap Draw Latch:15 ↔ bumper bracket - Copy:10
- [Mate]: 1872A111_Slide-Snap Draw Latch:15 ↔ bumper bracket - Copy:10
- [Mate]: bumper beam:6 ↔ 1872A111_Slide-Snap Draw Latch:15
- [Mate]: bumper beam:6 ↔ bumper bracket - Copy:10
- Mate:348: Chassis side 1:1 ↔ bumper piece 1:5
- Mate:349: Chassis side 1:1 ↔ bumper piece 1:5
- Mate:350: Chassis side 1:1 ↔ bumper beam:5
- Mate:351: Chassis side 1:1 ↔ bumper piece 1:6
- Mate:352: Chassis side 1:1 ↔ bumper piece 1:6
- Mate:353: Chassis side 1:1 ↔ bumper beam:6
- Mate:354: bumper simple:1 ↔ bumper bracket - Copy:8
- Mate:355: bumper simple:1 ↔ bumper bracket - Copy:9
- Mate:356: bumper simple:1 ↔ bumper bracket - Copy:10
- Mate:357: bumper simple:1 ↔ bumper bracket - Copy:6
- Mate:358: bumper simple:1 ↔ bumper bracket - Copy:7
- Mate:359: am-0940b 6 in HiGrip Wheel:10 ↔ am-2568 500EX Hex Hub:9
- Mate:360: am-0940b 6 in HiGrip Wheel:10 ↔ am-2568 500EX Hex Hub:9
- Mate:361: am-0940b 6 in HiGrip Wheel:10 ↔ am-2568 500EX Hex Hub:9
- Mate:362: WCP-0235:1 ↔ am-2568 500EX Hex Hub:9
- Mate:363: 217-3875-STEP-20140818:17 ↔ am-2568 500EX Hex Hub:9
- Mate:364: WCP-0235:1 ↔ am-2568 500EX Hex Hub:9
- [Mate]: am-0940b 6 in HiGrip Wheel:11 ↔ am-2568 500EX Hex Hub:10
- [Mate]: am-0940b 6 in HiGrip Wheel:11 ↔ am-2568 500EX Hex Hub:10
- [Mate]: am-0940b 6 in HiGrip Wheel:11 ↔ am-2568 500EX Hex Hub:10
- [Mate]: am-0940b 6 in HiGrip Wheel:12 ↔ am-2568 500EX Hex Hub:11
- [Mate]: am-0940b 6 in HiGrip Wheel:12 ↔ am-2568 500EX Hex Hub:11
- [Mate]: am-0940b 6 in HiGrip Wheel:12 ↔ am-2568 500EX Hex Hub:11
- [Mate]: am-0940b 6 in HiGrip Wheel:13 ↔ am-2568 500EX Hex Hub:12
- [Mate]: am-0940b 6 in HiGrip Wheel:13 ↔ am-2568 500EX Hex Hub:12
- [Mate]: am-0940b 6 in HiGrip Wheel:13 ↔ am-2568 500EX Hex Hub:12
- [Mate]: am-0940b 6 in HiGrip Wheel:14 ↔ am-2568 500EX Hex Hub:13
- [Mate]: am-0940b 6 in HiGrip Wheel:14 ↔ am-2568 500EX Hex Hub:13
- [Mate]: am-0940b 6 in HiGrip Wheel:14 ↔ am-2568 500EX Hex Hub:13
- Mate:377: drive hex shaft:4 ↔ am-2568 500EX Hex Hub:11
- Mate:378: drive hex shaft:4 ↔ am-2568 500EX Hex Hub:11
- Mate:379: 217-3875-STEP-20140818:12 ↔ am-2568 500EX Hex Hub:11
- Mate:380: drive hex shaft:5 ↔ am-2568 500EX Hex Hub:10
- Mate:381: drive hex shaft:5 ↔ am-2568 500EX Hex Hub:10
- Mate:382: 217-3875-STEP-20140818:13 ↔ am-2568 500EX Hex Hub:10
- Mate:383: drive hex shaft:6 ↔ am-2568 500EX Hex Hub:12
- Mate:384: drive hex shaft:6 ↔ am-2568 500EX Hex Hub:12
- Mate:385: 217-3875-STEP-20140818:11 ↔ am-2568 500EX Hex Hub:12
- Mate:386: drive hex shaft:3 ↔ am-2568 500EX Hex Hub:13
- Mate:387: drive hex shaft:3 ↔ am-2568 500EX Hex Hub:13
- Mate:388: 217-3875-STEP-20140818:5 ↔ am-2568 500EX Hex Hub:13
- [Mate]: am-0940b 6 in HiGrip Wheel:15 ↔ am-2568 500EX Hex Hub:14
- [Mate]: am-0940b 6 in HiGrip Wheel:15 ↔ am-2568 500EX Hex Hub:14
- [Mate]: am-0940b 6 in HiGrip Wheel:15 ↔ am-2568 500EX Hex Hub:14
- [Mate]: am-0940b 6 in HiGrip Wheel:16 ↔ am-2568 500EX Hex Hub:15
- [Mate]: am-0940b 6 in HiGrip Wheel:16 ↔ am-2568 500EX Hex Hub:15
- [Mate]: am-0940b 6 in HiGrip Wheel:16 ↔ am-2568 500EX Hex Hub:15
- [Mate]: am-0940b 6 in HiGrip Wheel:17 ↔ am-2568 500EX Hex Hub:16
- [Mate]: am-0940b 6 in HiGrip Wheel:17 ↔ am-2568 500EX Hex Hub:16
- [Mate]: am-0940b 6 in HiGrip Wheel:17 ↔ am-2568 500EX Hex Hub:16
- Mate:398: drive hex shaft:1 ↔ am-2568 500EX Hex Hub:15
- Mate:399: drive hex shaft:1 ↔ am-2568 500EX Hex Hub:15
- Mate:400: 217-3875-STEP-20140818:16 ↔ am-2568 500EX Hex Hub:15
- Mate:401: WCP-0235:2 ↔ am-2568 500EX Hex Hub:14
- Mate:402: WCP-0235:2 ↔ am-2568 500EX Hex Hub:14
- Mate:403: 217-3875-STEP-20140818:18 ↔ am-2568 500EX Hex Hub:14
- Mate:404: drive hex shaft:2 ↔ am-2568 500EX Hex Hub:16
- Mate:405: drive hex shaft:2 ↔ am-2568 500EX Hex Hub:16
- Mate:406: 217-3875-STEP-20140818:3 ↔ am-2568 500EX Hex Hub:16
- Flush:17: drive hex shaft:6 ↔ TTB-0013_Balanced Half Inch Hex Shaft Collar:11
- Flush:18: drive hex shaft:5 ↔ TTB-0013_Balanced Half Inch Hex Shaft Collar:9
- Flush:19: drive hex shaft:4 ↔ TTB-0013_Balanced Half Inch Hex Shaft Collar:7
- Mate:407: Chassis side 2:2 ↔ TTB-00012_T-Gusset:2
- Mate:408: Chassis side 2:2 ↔ TTB-00012_T-Gusset:9
- Mate:409: Chassis side 2:2 ↔ TTB-00012_T-Gusset:9
- Mate:410: Chassis side 1:2 ↔ TTB-00012_T-Gusset:9
- Mate:411: Chassis side 1:2 ↔ Robot bottom:1
- Mate:412: bumper simple:1 ↔ Robot bottom:1
- Mate:413 (25.4 mm): am-3000a National Instruments roboRIO 2:1 ↔ Robot bottom:1
- Mate:415: Robot bottom:1 ↔ REV-11-1850:1
- Mate:416: Robot bottom:1 ↔ REV-11-1852:1
- Mate:417: Robot bottom:1 ↔ am-0282 120a Circuit Breaker:1
- Mate:418 (25.4 mm): am-3227 Pneumatic Compressor 1.1_Pump REV2:1 ↔ Robot bottom:1
- [Mate]: 217-3875-STEP-20140818:22 ↔ intake-1:2
- [Mate]: 217-3875-STEP-20140818:22 ↔ intake-1:2
- [Mate]: 217-3875-STEP-20140818:23 ↔ intake-1:2
- [Mate]: 217-3875-STEP-20140818:23 ↔ intake-1:2
- Mate:431: 217-3875-STEP-20140818:22 ↔ Intake hex:1
- Mate:432: 217-3875-STEP-20140818:22 ↔ Intake hex:1
- Mate:433: 217-3875-STEP-20140818:23 ↔ Intake hex:2
- Mate:434: TTB-0058 5M 15t HTD ALUMINUM PULLEY:1 ↔ Intake hex:2
- Mate:435: TTB-0058 5M 15t HTD ALUMINUM PULLEY:1 ↔ Intake hex:2
- Mate:436: TTB-0058 5M 15t HTD ALUMINUM PULLEY:2 ↔ Intake hex:1
- Mate:437: TTB-0058 5M 15t HTD ALUMINUM PULLEY:2 ↔ Intake hex:1
- Mate:438: TTB-0058 5M 15t HTD ALUMINUM PULLEY:2 ↔ 217-3875-STEP-20140818:22
- Mate:439: TTB-0058 5M 15t HTD ALUMINUM PULLEY:1 ↔ 217-3875-STEP-20140818:23
- Mate:440: TTB-0013_Balanced Half Inch Hex Shaft Collar:12 ↔ Intake hex:2
- Mate:441: TTB-0013_Balanced Half Inch Hex Shaft Collar:12 ↔ Intake hex:2
- Flush:20: TTB-0013_Balanced Half Inch Hex Shaft Collar:12 ↔ Intake hex:2
- Mate:442: TTB-0013_Balanced Half Inch Hex Shaft Collar:13 ↔ Intake hex:1
- Mate:443: TTB-0013_Balanced Half Inch Hex Shaft Collar:13 ↔ Intake hex:1
- Flush:21: TTB-0013_Balanced Half Inch Hex Shaft Collar:13 ↔ Intake hex:1
- Mate:444: TTB-0013_Balanced Half Inch Hex Shaft Collar:13 ↔ TTB-0058 5M 15t HTD ALUMINUM PULLEY:2
- Mate:445: TTB-0013_Balanced Half Inch Hex Shaft Collar:12 ↔ TTB-0058 5M 15t HTD ALUMINUM PULLEY:1
- Mate:465: 1872A111_Slide-Snap Draw Latch:9 ↔ bumper bracket - Copy:4
- Mate:469: 217-3875-STEP-20140818:23 ↔ Intake hex:2
- Mate:472: TTB-0013_Balanced Half Inch Hex Shaft Collar:12 ↔ 217-3875-STEP-20140818:23
- Mate:473: Intake hex:1 ↔ am-4541 Sushi Roller 500 Hex Bore:23
- Mate:474: Intake hex:1 ↔ am-4541 Sushi Roller 500 Hex Bore:23
- Mate:475: 217-3875-STEP-20140818:22 ↔ am-4541 Sushi Roller 500 Hex Bore:23
- Mate:476: Intake hex:1 ↔ am-3480 4IN 500Hex Bore Compliant Wheel REV2:8
- Mate:477: Intake hex:1 ↔ am-3480 4IN 500Hex Bore Compliant Wheel REV2:8
- Mate:478: am-3480 4IN 500Hex Bore Compliant Wheel REV2:8 ↔ am-4541 Sushi Roller 500 Hex Bore:23
- Mate:479: 217-3875-STEP-20140818:24 ↔ intake-1:3
- Mate:480: 217-3875-STEP-20140818:25 ↔ intake-1:3
- Mate:481: 217-3875-STEP-20140818:25 ↔ intake-1:3
- Mate:482: 217-3875-STEP-20140818:24 ↔ intake-1:3
- Mate:483: 217-3875-STEP-20140818:24 ↔ Intake hex:1
- Mate:484: 217-3875-STEP-20140818:25 ↔ Intake hex:2
- Mate:485: 217-3875-STEP-20140818:25 ↔ Intake hex:2
- Mate:486: 217-3875-STEP-20140818:25 ↔ intake-1:3
- Mate:487: 217-3875-STEP-20140818:25 ↔ intake-1:3
- Mate:490: TTB-0013_Balanced Half Inch Hex Shaft Collar:15 ↔ Intake hex:2
- Mate:491: TTB-0013_Balanced Half Inch Hex Shaft Collar:15 ↔ Intake hex:2
- Mate:492: am-4541 Sushi Roller 500 Hex Bore:32 ↔ Intake hex:1
- Mate:493: am-4541 Sushi Roller 500 Hex Bore:32 ↔ Intake hex:1
- Mate:494: am-4541 Sushi Roller 500 Hex Bore:32 ↔ am-3480 4IN 500Hex Bore Compliant Wheel REV2:32
- Mate:495: am-4541 Sushi Roller 500 Hex Bore:32 ↔ 217-3875-STEP-20140818:24
- Mate:496: 217-3875-STEP-20140818:25 ↔ Intake hex:2
- Mate:497: TTB-0013_Balanced Half Inch Hex Shaft Collar:16 ↔ Intake hex:1
- Mate:498: TTB-0013_Balanced Half Inch Hex Shaft Collar:16 ↔ Intake hex:1
- Mate:499: TTB-0013_Balanced Half Inch Hex Shaft Collar:16 ↔ 217-3875-STEP-20140818:24
- Mate:500: TTB-0013_Balanced Half Inch Hex Shaft Collar:15 ↔ 217-3875-STEP-20140818:25
- Mate:501: am-4541 Sushi Roller 500 Hex Bore:32 ↔ intake-1:3
- Mate:502: Intake hex:2 ↔ am-4541 Sushi Roller 500 Hex Bore:33
- Mate:503: Intake hex:2 ↔ am-4541 Sushi Roller 500 Hex Bore:33
- Mate:504: Intake hex:2 ↔ am-3480 4IN 500Hex Bore Compliant Wheel REV2:33
- Mate:505: Intake hex:2 ↔ am-3480 4IN 500Hex Bore Compliant Wheel REV2:33
- Mate:506: am-4541 Sushi Roller 500 Hex Bore:33 ↔ am-3480 4IN 500Hex Bore Compliant Wheel REV2:33
- Mate:507: intake-1:2 ↔ am-4541 Sushi Roller 500 Hex Bore:33
- Mate:508: am-4541 Sushi Roller 500 Hex Bore:2 ↔ Intake hex:2
- Mate:509: am-4541 Sushi Roller 500 Hex Bore:2 ↔ Intake hex:2
- Mate:510: am-4541 Sushi Roller 500 Hex Bore:2 ↔ intake-1:3
- Mate:511: 217-3875-STEP-20140818:24 ↔ Intake hex:1
- Mate:512: 217-3875-STEP-20140818:24 ↔ intake-1:3
- Flush:22 (11.43 mm): TTB-0013_Balanced Half Inch Hex Shaft Collar:16 ↔ Intake hex:1
- Mate:513: 217-3875-STEP-20140818:23 ↔ Intake hex:2
- Mate:514: Intake mount:1 ↔ TTB-00012_T-Gusset:6
- Mate:515: Intake mount:1 ↔ TTB-00012_T-Gusset:6
- Mate:516: Intake mount:1 ↔ TTB-00012_T-Gusset:6
- Mate:517: Intake mount:2 ↔ TTB-00012_T-Gusset:2
- Mate:518: Intake mount:2 ↔ TTB-00012_T-Gusset:2
- Mate:519: Intake mount:2 ↔ TTB-00012_T-Gusset:2
- Mate:520: 217-3875-STEP-20140818:26 ↔ Intake mount:1
- Mate:521: 217-3875-STEP-20140818:27 ↔ Intake mount:1
- Mate:522: 217-3875-STEP-20140818:27 ↔ Intake mount:1
- Mate:523: 217-3875-STEP-20140818:26 ↔ Intake mount:1
- Mate:524: 217-3875-STEP-20140818:28 ↔ Intake mount:2
- Mate:525: 217-3875-STEP-20140818:29 ↔ Intake mount:2
- Mate:526: 217-3875-STEP-20140818:29 ↔ Intake mount:2
- Mate:527: 217-3875-STEP-20140818:28 ↔ Intake mount:2
- Mate:528: 217-3875-STEP-20140818:30 ↔ intake-1:2
- Mate:529: 217-3875-STEP-20140818:30 ↔ intake-1:2
- Mate:530: 217-3875-STEP-20140818:31 ↔ intake-1:3
- Mate:531: 217-3875-STEP-20140818:31 ↔ intake-1:3
- Mate:532: Intake base hex:1 ↔ 217-3875-STEP-20140818:31
- Mate:533: Intake base hex:1 ↔ 217-3875-STEP-20140818:31
- Mate:534: Intake base hex:1 ↔ 217-3875-STEP-20140818:30
- Mate:535: Intake base hex:1 ↔ 217-3875-STEP-20140818:28
- Mate:536: Intake base hex:1 ↔ 217-3875-STEP-20140818:28
- Mate:537: Intake mount:1 ↔ intake-1:3
## Named parameters: d94_d88 = 0 mm, d95_d89 = 0 mm, d96_d90 = 0 mm, d97_d88 = 0 mm, d98_d89 = 0 mm, d99_d90 = 0 mm, d109_d106 = 0 mm, d110_d107 = 0 mm, d111_d108 = 0 mm, d118_d106 = 0 mm, d119_d107 = 0 mm, d120_d108 = 0 mm, d165_d126 = 0 mm, d166_d127 = 0 mm, d167_d132 = 0 mm, d168_d133 = 0 mm, d169_d134 = 0 mm, d170_d135 = 0 mm, d171_d136 = 0 mm, d172_d143 = 0 mm, d184_d164 = 0 mm, d185_d126 = 0 mm, d186_d127 = 0 mm, d187_d132 = 0 mm, d188_d133 = 0 mm, d189_d134 = 0 mm, d190_d135 = 0 mm, d191_d136 = 0 mm, d192_d143 = 0 mm, d204_d164 = 0 mm, d205_d126 = 0 mm, d206_d127 = 0 mm, d207_d132 = 0 mm, d208_d133 = 0 mm, d209_d134 = 0 mm, d210_d135 = 0 mm, d211_d136 = 0 mm, d212_d143 = 0 mm, d224_d164 = 0 mm, d238_d205_d126 = 0 mm, d239_d206_d127 = 0 mm, d240_d207_d132 = 0 mm, d241_d208_d133 = 0 mm, d242_d209_d134 = 0 mm, d243_d210_d135 = 0 mm, d244_d211_d136 = 0 mm, d245_d212_d143 = 0 mm, d257_d224_d164 = 0 mm, d258_d205_d126 = 0 mm, d259_d206_d127 = 0 mm, d260_d207_d132 = 0 mm, d261_d208_d133 = 0 mm, d262_d209_d134 = 0 mm, d263_d210_d135 = 0 mm, d264_d211_d136 = 0 mm, d265_d212_d143 = 0 mm, d277_d224_d164 = 0 mm, d332_d109_d106 = 0 mm, d333_d110_d107 = 0 mm, d334_d111_d108 = 0 mm, d338_d335 = 0 mm, d339_d336 = 0 mm, d340_d327 = 0 mm, d341_d331 = 0 mm, d342_d332_d109_d106 = 0 mm, d343_d333_d110_d107 = 0 mm, d344_d334_d111_d108 = 0 mm, d345_d335 = 0 mm, d346_d336 = 0 mm, d347_d327 = 0 mm, d348_d331 = 0 mm, d349_d332_d109_d106 = 0 mm, d350_d333_d110_d107 = 0 mm, d351_d334_d111_d108 = 0 mm, d352_d335 = 0 mm, d353_d336 = 0 mm, d354_d327 = 0 mm, d355_d331 = 0 mm, d356_d332_d109_d106 = 0 mm, d357_d333_d110_d107 = 0 mm, d358_d334_d111_d108 = 0 mm, d368_d352_d335 = 0 mm, d369_d353_d336 = 0 mm, d370_d354_d327 = 0 mm, d371_d355_d331 = 0 mm, d372_d356_d332_d109_d106 = 0 mm, d373_d357_d333_d110_d107 = 0 mm, d374_d358_d334_d111_d108 = 0 mm, d375_d352_d335 = 0 mm, d376_d353_d336 = 0 mm, d377_d354_d327 = 0 mm, d378_d355_d331 = 0 mm, d379_d356_d332_d109_d106 = 0 mm, d380_d357_d333_d110_d107 = 0 mm, d381_d358_d334_d111_d108 = 0 mm, d399_d393 = 0 mm, d400_d394 = 0 mm, d401_d395 = 0 mm, d402_d393 = 0 mm, d403_d394 = 0 mm, d404_d395 = 0 mm, d405_d393 = 0 mm, d406_d394 = 0 mm, d407_d395 = 0 mm, d408_d393 = 0 mm, d409_d394 = 0 mm, d410_d395 = 0 mm, d423_d408_d393 = 0 mm, d424_d409_d394 = 0 mm, d425_d410_d395 = 0 mm, d426_d408_d393 = 0 mm, d427_d409_d394 = 0 mm, d428_d410_d395 = 0 mm, d429_d408_d393 = 0 mm, d430_d409_d394 = 0 mm, d431_d410_d395 = 0 mm, d465_d457 = 0 mm, d466_d458 = 0 mm, d467_d459 = 0 mm, d468_d460 = 0 mm
